# Autodesk Inventor assembly: rs775_4
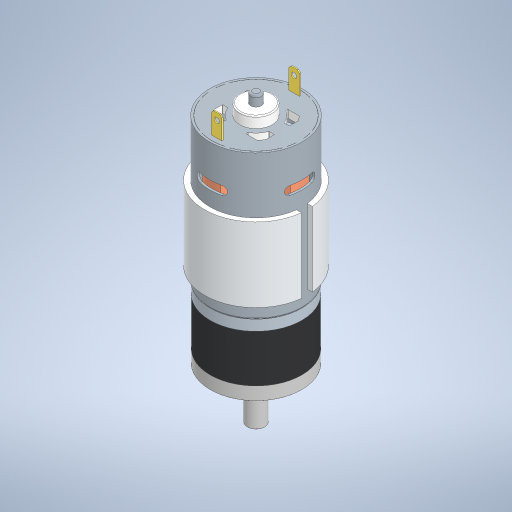
[picture p0: Inventor's stored thumbnail of the model, 512x512]
Saved by Autodesk Inventor 2024.2 (Build 282272000, 272)
## iProperties
Created: 2023-12-04
Part Number: rs775_4
Document SubType Name: Assembly
Designer: fhbdh
Author: fhbdh
## Documents named in this file (3)
- C:\Users\fhbdh\OneDrive - Kyushu University\ドキュメント\ロボコン\2024_ABU\machine_2024_ABU\omuni_wheel\parts\frequently used parts\モーター\RS775\rs775_4.iam
- C:\Users\fhbdh\OneDrive - Kyushu University\ドキュメント\ロボコン\2024_ABU\machine_2024_ABU\omuni_wheel\parts\frequently used parts\モーター\RS775\775_moter.ipt
- C:\Users\fhbdh\OneDrive - Kyushu University\ドキュメント\ロボコン\2024_ABU\machine_2024_ABU\omuni_wheel\parts\frequently used parts\モーター\RS775\IG42C-004-D8.ipt
## Components (2 placed, 2 different names)
1. 775_moter:1 — 挿入:1, 挿入:2
2. IG42C-004-D8:1 — 挿入:1, 挿入:2
## Relationships (2: Insert 2)
- 挿入:1 [Insert]: 775_moter:1 ↔ IG42C-004-D8:1
- 挿入:2 [Insert]: 775_moter:1 ↔ IG42C-004-D8:1
